# Autodesk Inventor assembly: electronics
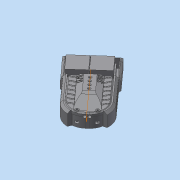
[picture p0: Inventor's stored thumbnail of the model, 180x180]
Saved by Autodesk Inventor 2014 SP1 (Build 180222100, 222)
## iProperties
Created: 2014-05-24
Part Number: electronics
Document SubType Name: Assembly
Designer: brent
Author: brent
## Documents named in this file (4)
- C:\Users\brent\Documents\electric-longboard\brent\electronics.iam
- C:\Users\brent\Documents\electric-longboard\brent\electronicsbox_top.ipt
- C:\Users\brent\Documents\electric-longboard\brent\electronicsbox_lid.ipt
- C:\Users\brent\Documents\electric-longboard\brent\hobbyking150acaresc.ipt
## Components (4 placed, 3 different names)
1. electronicsbox_top:1 — Mate:4, Mate:5, Mate:6, Mate:7, Mate:8, Mate:9, Mate:18
2. electronicsbox_lid:1 — Mate:4, Mate:5, Mate:18
3. hobbyking150acaresc:1 — Mate:6, Mate:8
4. hobbyking150acaresc:2 — Mate:7, Mate:9
## Relationships (7: Mate 7)
- Mate:4: electronicsbox_top:1 ↔ electronicsbox_lid:1
- Mate:5: electronicsbox_top:1 ↔ electronicsbox_lid:1
- Mate:6: electronicsbox_top:1 ↔ hobbyking150acaresc:1
- Mate:7: electronicsbox_top:1 ↔ hobbyking150acaresc:2
- Mate:8 (3.81 mm): electronicsbox_top:1 ↔ hobbyking150acaresc:1
- Mate:9 (3.81 mm): electronicsbox_top:1 ↔ hobbyking150acaresc:2
- Mate:18 (1.27 mm): electronicsbox_top:1 ↔ electronicsbox_lid:1
